# Autodesk Inventor assembly: SirHexAlot
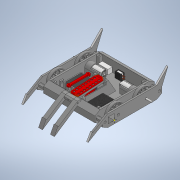
[picture p0: Inventor's stored thumbnail of the model, 180x180]
Saved by Autodesk Inventor 2020 (Build 240168000, 168)
## iProperties
Created: 2023-12-21
Part Number: SirHexAlot
Document SubType Name: Assembly
Designer: smz3rm
Mass: 451.68 g
Surface Area: 1749 cm^2
Volume: 353.403 cm^3
Density: 1.27809 g/cm^3
Author: smz3rm
## Documents named in this file (21)
- C:\Users\smz3rm\OneDrive - BP\Documents\DigitalTwin\Models\BattleBot\Flipper\SirHexAlot.iam
- C:\Users\smz3rm\OneDrive - BP\Documents\DigitalTwin\Models\BattleBot\Flipper\HexBody.ipt
- C:\Users\smz3rm\OneDrive - BP\Documents\DigitalTwin\Models\BattleBot\Flipper\PulleyedWheelV1.ipt
- C:\Users\smz3rm\OneDrive - BP\Documents\DigitalTwin\Models\BattleBot\DriveMotorV2.ipt
- C:\Users\smz3rm\OneDrive - BP\Documents\DigitalTwin\Models\BattleBot\SwitchHolder.ipt
- C:\Users\smz3rm\OneDrive - BP\Documents\DigitalTwin\Models\BattleBot\Switch.ipt
- C:\Users\smz3rm\OneDrive - BP\Documents\DigitalTwin\Models\BattleBot\BatteryV1.ipt
- C:\Users\smz3rm\OneDrive - BP\Documents\DigitalTwin\Models\BattleBot\Flipper\Servo.ipt
- C:\Users\smz3rm\OneDrive - BP\Documents\DigitalTwin\Models\BattleBot\Flipper\PulleyedBearingWheelV1.ipt
- C:\Users\smz3rm\OneDrive - BP\Documents\DigitalTwin\Models\BattleBot\Flipper\WheelBearings.ipt
- C:\Users\smz3rm\OneDrive - BP\Documents\DigitalTwin\Models\BattleBot\Flipper\FlipperRod.ipt
- C:\Users\smz3rm\OneDrive - BP\Documents\DigitalTwin\Models\BattleBot\Flipper\HexFlipper.ipt
- C:\Users\smz3rm\OneDrive - BP\Documents\DigitalTwin\Models\BattleBot\Flipper\HexFlipperSpike.ipt
- C:\Users\smz3rm\OneDrive - BP\Documents\DigitalTwin\Models\BattleBot\Flipper\HexWheelGuardLeft.ipt
- C:\Users\smz3rm\OneDrive - BP\Documents\DigitalTwin\Models\BattleBot\Flipper\HexWheelGuardRight.ipt
- C:\Users\smz3rm\OneDrive - BP\Documents\DigitalTwin\Models\BattleBot\FS2A.ipt
- C:\Users\smz3rm\OneDrive - BP\Documents\DigitalTwin\Models\BattleBot\Flipper\HexFlipperArmConnector.ipt
- C:\Users\smz3rm\OneDrive - BP\Documents\DigitalTwin\Models\BattleBot\Flipper\ServoArm.ipt
- C:\Users\smz3rm\OneDrive - BP\Documents\DigitalTwin\Models\BattleBot\Flipper\HexServoCover.ipt
- C:\Users\smz3rm\OneDrive - BP\Documents\DigitalTwin\Models\BattleBot\Flipper\HexSideSpike.ipt
- C:\Users\smz3rm\OneDrive - BP\Documents\DigitalTwin\Models\BattleBot\Flipper\HexFlipperRigid.ipt
## Components (28 placed, 20 different names)
1. HexBody:1 — Mate:4, Mate:5, Mate:7, Mate:8, Mate:11, Mate:14, Mate:22, Mate:24, Mate:39, Mate:41, Mate:42, Mate:48, Mate:51, Mate:62, Flush:1, Mate:63, Mate:64, Mate:67, Mate:68, Mate:69, Mate:72, Mate:73, Mate:80, Mate:82, Mate:83, Flush:3, Mate:91, Mate:95, Mate:96, Mate:97, Mate:98, Mate:99, Mate:100, Mate:102, Mate:103, Mate:106
2. PulleyedWheelV1:1 — Mate:10, Mate:11
3. DriveMotorV2:1 — Mate:7, Mate:8, Mate:10, Mate:65, Mate:103
4. DriveMotorV2:2 — Mate:4, Mate:5, Mate:15, Mate:70, Mate:102
5. SwitchHolder:1 — Mate:19, Mate:20, Mate:21, Mate:22, Mate:95
6. Switch:1 — Mate:19, Mate:20, Mate:21
7. BatteryV1:1 — Mate:24, Mate:97, Mate:98
8. PulleyedWheelV1:5 — Mate:14, Mate:15
9. Servo:1 — Mate:83, Mate:84, Mate:85, Mate:91, Mate:101
10. PulleyedBearingWheelV1:1 — Mate:31, Mate:32, Mate:33, Mate:42
11. PulleyedBearingWheelV1:2 — Mate:35, Mate:37, Mate:38, Mate:39, Mate:72
12. WheelBearings:1 — Mate:31, Mate:32, Mate:66
13. WheelBearings:2 — Mate:33, Mate:41
14. WheelBearings:3 — Mate:35
15. WheelBearings:4 — Mate:37, Mate:38, Mate:71
16. FlipperRod:1 — Mate:49, Mate:50
17. HexFlipper:1 — Mate:49, Mate:50, Mate:51, Mate:62, Mate:74, Mate:75, Mate:76, Mate:77, Mate:78, Mate:79, Flush:2, Mate:89, Mate:90, Mate:110, Mate:111, Flush:4
18. HexFlipperSpike:1 — Mate:77, Mate:78, Mate:79, Mate:93
19. HexFlipperSpike:2 — Mate:74, Mate:75, Mate:76, Mate:94
20. HexWheelGuardLeft:1 — Mate:63, Mate:64, Mate:65, Mate:66, Mate:67, Mate:92, Mate:104, Mate:105, Mate:108
21. HexWheelGuardRight:1 — Mate:68, Mate:69, Mate:70, Mate:71, Mate:73, Mate:109
22. FS2A:1 — Mate:80, Mate:82, Mate:96
23. HexFlipperArmConnector:1 — Mate:87, Mate:89, Mate:90
24. ServoArm:1 — Mate:84, Mate:85, Flush:2, Mate:87
25. HexServoCover:1 — Mate:99, Mate:100, Mate:101
26. HexSideSpike:2 — Mate:108
27. HexSideSpike:4 — Mate:109
28. HexFlipperRigid:1 — Mate:110, Mate:111, Flush:4
## Relationships (76: Mate 72, Flush 4)
- Mate:4: HexBody:1 ↔ DriveMotorV2:2
- Mate:5: HexBody:1 ↔ DriveMotorV2:2
- Mate:7: HexBody:1 ↔ DriveMotorV2:1
- Mate:8: HexBody:1 ↔ DriveMotorV2:1
- Mate:10: PulleyedWheelV1:1 ↔ DriveMotorV2:1
- Mate:11: HexBody:1 ↔ PulleyedWheelV1:1
- Mate:14: HexBody:1 ↔ PulleyedWheelV1:5
- Mate:15: DriveMotorV2:2 ↔ PulleyedWheelV1:5
- Mate:19: SwitchHolder:1 ↔ Switch:1
- Mate:20: SwitchHolder:1 ↔ Switch:1
- Mate:21: SwitchHolder:1 ↔ Switch:1
- Mate:22: HexBody:1 ↔ SwitchHolder:1
- Mate:24: HexBody:1 ↔ BatteryV1:1
- Mate:31: PulleyedBearingWheelV1:1 ↔ WheelBearings:1
- Mate:32: PulleyedBearingWheelV1:1 ↔ WheelBearings:1
- Mate:33: PulleyedBearingWheelV1:1 ↔ WheelBearings:2
- Mate:35: PulleyedBearingWheelV1:2 ↔ WheelBearings:3
- Mate:37: PulleyedBearingWheelV1:2 ↔ WheelBearings:4
- Mate:38: PulleyedBearingWheelV1:2 ↔ WheelBearings:4
- Mate:39: HexBody:1 ↔ PulleyedBearingWheelV1:2
- Mate:41: HexBody:1 ↔ WheelBearings:2
- Mate:42: HexBody:1 ↔ PulleyedBearingWheelV1:1
- Mate:48: HexBody:1
- Mate:49: FlipperRod:1 ↔ HexFlipper:1
- Mate:50: FlipperRod:1 ↔ HexFlipper:1
- Mate:51: HexBody:1 ↔ HexFlipper:1
- Mate:62 (1 mm): HexBody:1 ↔ HexFlipper:1
- Flush:1: HexBody:1
- Mate:63: HexBody:1 ↔ HexWheelGuardLeft:1
- Mate:64: HexBody:1 ↔ HexWheelGuardLeft:1
- Mate:65: DriveMotorV2:1 ↔ HexWheelGuardLeft:1
- Mate:66: WheelBearings:1 ↔ HexWheelGuardLeft:1
- Mate:67: HexBody:1 ↔ HexWheelGuardLeft:1
- Mate:68: HexBody:1 ↔ HexWheelGuardRight:1
- Mate:69: HexBody:1 ↔ HexWheelGuardRight:1
- Mate:70: DriveMotorV2:2 ↔ HexWheelGuardRight:1
- Mate:71: WheelBearings:4 ↔ HexWheelGuardRight:1
- Mate:72: HexBody:1 ↔ PulleyedBearingWheelV1:2
- Mate:73: HexBody:1 ↔ HexWheelGuardRight:1
- Mate:74: HexFlipper:1 ↔ HexFlipperSpike:2
- Mate:75: HexFlipper:1 ↔ HexFlipperSpike:2
- Mate:76: HexFlipper:1 ↔ HexFlipperSpike:2
- Mate:77: HexFlipper:1 ↔ HexFlipperSpike:1
- Mate:78: HexFlipper:1 ↔ HexFlipperSpike:1
- Mate:79: HexFlipper:1 ↔ HexFlipperSpike:1
- Mate:80: HexBody:1 ↔ FS2A:1
- Mate:82: HexBody:1 ↔ FS2A:1
- Mate:83: HexBody:1 ↔ Servo:1
- Mate:84: Servo:1 ↔ ServoArm:1
- Mate:85: Servo:1 ↔ ServoArm:1
- Flush:2: HexFlipper:1 ↔ ServoArm:1
- Mate:87: HexFlipperArmConnector:1 ↔ ServoArm:1
- Mate:89: HexFlipper:1 ↔ HexFlipperArmConnector:1
- Flush:3: HexBody:1
- Mate:90: HexFlipper:1 ↔ HexFlipperArmConnector:1
- Mate:91: HexBody:1 ↔ Servo:1
- Mate:92: HexWheelGuardLeft:1
- Mate:93: HexFlipperSpike:1
- Mate:94: HexFlipperSpike:2
- Mate:95: HexBody:1 ↔ SwitchHolder:1
- Mate:96: HexBody:1 ↔ FS2A:1
- Mate:97: HexBody:1 ↔ BatteryV1:1
- Mate:98: HexBody:1 ↔ BatteryV1:1
- Mate:99: HexBody:1 ↔ HexServoCover:1
- Mate:100: HexBody:1 ↔ HexServoCover:1
- Mate:101: Servo:1 ↔ HexServoCover:1
- Mate:102: HexBody:1 ↔ DriveMotorV2:2
- Mate:103: HexBody:1 ↔ DriveMotorV2:1
- Mate:104: HexWheelGuardLeft:1
- Mate:105: HexWheelGuardLeft:1
- Mate:106: HexBody:1
- Mate:108: HexWheelGuardLeft:1 ↔ HexSideSpike:2
- Mate:109: HexWheelGuardRight:1 ↔ HexSideSpike:4
- Mate:110: HexFlipper:1 ↔ HexFlipperRigid:1
- Mate:111: HexFlipper:1 ↔ HexFlipperRigid:1
- Flush:4: HexFlipper:1 ↔ HexFlipperRigid:1
